# Autodesk Inventor assembly: CLB_089_ClimberMount
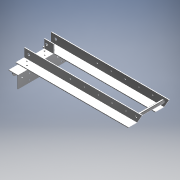
[picture p0: Inventor's stored thumbnail of the model, 180x180]
Saved by Autodesk Inventor 2018.3 (Build 223284000, 284)
## iProperties
Created: 2020-02-22
Part Number: CLB_089_ClimberMount
Document SubType Name: Assembly
Designer: 22perngrac
Mass: 823.096 g
Surface Area: 2005.18 cm^2
Volume: 304.85 cm^3
Density: 2.7 g/cm^3
Author: 22perngrac
## Documents named in this file (7)
- C:\Users\22perngrac\Documents\GrabCAD\Infinite Recharge 2020\Build season\CLB_089_ClimberMount.iam
- C:\Users\22perngrac\Documents\GrabCAD\Infinite Recharge 2020\Build season\CLB_088_ClimberMountBar.ipt
- C:\Users\22perngrac\Documents\GrabCAD\Infinite Recharge 2020\Build season\CLB_087_ClimberMountBracketGusset.ipt
- C:\Users\22perngrac\Documents\GrabCAD\Infinite Recharge 2020\Build season\CLB_086_ClimberMountLowerAngle.ipt
- C:\Users\22perngrac\Documents\GrabCAD\Infinite Recharge 2020\Build season\CLB_085_ClimberMountLBracket.ipt
- C:\Users\22perngrac\Documents\GrabCAD\Infinite Recharge 2020\Build season\CLB_084_ClimberMountTopAngle.ipt
- C:\Users\22perngrac\Documents\GrabCAD\Infinite Recharge 2020\Build season\CLB_079_ClimberMountReinforceBar.ipt
## Components (8 placed, 6 different names)
1. CLB_088_ClimberMountBar:1 — Insert:1
2. CLB_087_ClimberMountBracketGusset:1 — Mate:4, Flush:7, Mate:5
3. CLB_087_ClimberMountBracketGusset:2 — Mate:6, Flush:8, Mate:7
4. CLB_086_ClimberMountLowerAngle:1 — Mate:1, Flush:1, Flush:2, Mate:2, Flush:3, Flush:4, Mate:3, Flush:5, Flush:6, Mate:8, Mate:9, Mate:10
5. CLB_085_ClimberMountLBracket:1 — Mate:3, Flush:5, Flush:6
6. CLB_084_ClimberMountTopAngle:1 — Mate:1, Flush:1, Flush:2, Mate:4, Flush:7, Mate:5
7. CLB_084_ClimberMountTopAngle:2 — Mate:2, Flush:3, Flush:4, Mate:6, Flush:8, Mate:7, Insert:1
8. CLB_079_ClimberMountReinforceBar:1 — Mate:8, Mate:9, Mate:10
## Relationships (19: Mate 10, Flush 8, Insert 1)
- Mate:1: CLB_086_ClimberMountLowerAngle:1 ↔ CLB_084_ClimberMountTopAngle:1
- Flush:1 (15.875 mm): CLB_086_ClimberMountLowerAngle:1 ↔ CLB_084_ClimberMountTopAngle:1
- Flush:2 (-9.525 mm): CLB_086_ClimberMountLowerAngle:1 ↔ CLB_084_ClimberMountTopAngle:1
- Mate:2: CLB_086_ClimberMountLowerAngle:1 ↔ CLB_084_ClimberMountTopAngle:2
- Flush:3 (-9.525 mm): CLB_086_ClimberMountLowerAngle:1 ↔ CLB_084_ClimberMountTopAngle:2
- Flush:4 (127 mm): CLB_086_ClimberMountLowerAngle:1 ↔ CLB_084_ClimberMountTopAngle:2
- Mate:3: CLB_086_ClimberMountLowerAngle:1 ↔ CLB_085_ClimberMountLBracket:1
- Flush:5: CLB_086_ClimberMountLowerAngle:1 ↔ CLB_085_ClimberMountLBracket:1
- Flush:6 (53.975 mm): CLB_086_ClimberMountLowerAngle:1 ↔ CLB_085_ClimberMountLBracket:1
- Mate:4: CLB_087_ClimberMountBracketGusset:1 ↔ CLB_084_ClimberMountTopAngle:1
- Flush:7 (127 mm): CLB_087_ClimberMountBracketGusset:1 ↔ CLB_084_ClimberMountTopAngle:1
- Mate:5: CLB_087_ClimberMountBracketGusset:1 ↔ CLB_084_ClimberMountTopAngle:1
- Mate:6: CLB_087_ClimberMountBracketGusset:2 ↔ CLB_084_ClimberMountTopAngle:2
- Flush:8 (127 mm): CLB_087_ClimberMountBracketGusset:2 ↔ CLB_084_ClimberMountTopAngle:2
- Mate:7: CLB_087_ClimberMountBracketGusset:2 ↔ CLB_084_ClimberMountTopAngle:2
- Insert:1: CLB_088_ClimberMountBar:1 ↔ CLB_084_ClimberMountTopAngle:2
- Mate:8: CLB_086_ClimberMountLowerAngle:1 ↔ CLB_079_ClimberMountReinforceBar:1
- Mate:9: CLB_086_ClimberMountLowerAngle:1 ↔ CLB_079_ClimberMountReinforceBar:1
- Mate:10 (25.4 mm): CLB_086_ClimberMountLowerAngle:1 ↔ CLB_079_ClimberMountReinforceBar:1
